# Autodesk Inventor assembly: ThighKneeGear
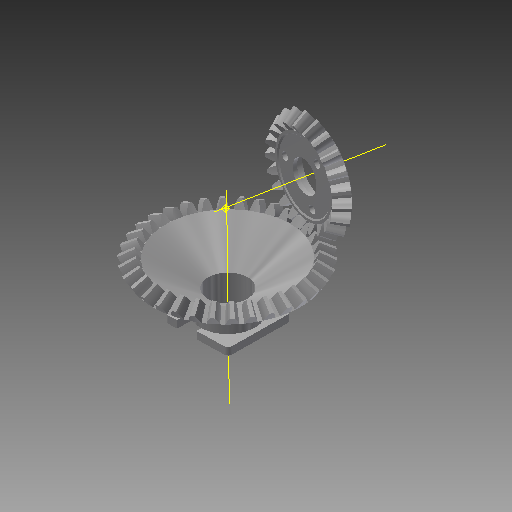
[picture p0: Inventor's stored thumbnail of the model, 512x512]
Saved by Autodesk Inventor 2018 (Build 220112000, 112)
## iProperties
Created: 2017-09-29
Part Number: ThighKneeGear
Material: Generisch
Document SubType Name: Assembly
Designer: JochenAlt
Author: JochenAlt
## Documents named in this file (3)
- D:\Projects\Manfred\design\cad\Inventor\ThighKneeGear.iam
- D:\Projects\Manfred\design\cad\Inventor\Kegelräder 040x\Konstruktions-Assistent\Kegelrad11.ipt
- D:\Projects\Manfred\design\cad\Inventor\Kegelräder 040x\Konstruktions-Assistent\Kegelrad21.ipt
## Components (2 placed, 2 different names)
1. Kegelrad1:1 — Passend:1, Winkel:1, Passend:2, Drehung:1
2. Kegelrad2:1 — Passend:1, Winkel:1, Passend:2, Drehung:1
## Relationships (4: Mate 2, Angle 1, RelateRotation 1)
- Passend:1 [Mate]: Kegelrad1:1 ↔ Kegelrad2:1
- Winkel:1 [Angle] (90 deg): Kegelrad1:1 ↔ Kegelrad2:1
- Passend:2 [Mate]: Kegelrad1:1 ↔ Kegelrad2:1
- Drehung:1 [RelateRotation] (1.65 ul): Kegelrad1:1 ↔ Kegelrad2:1
